# Autodesk Inventor assembly: s-assy-motor
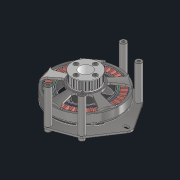
[picture p0: Inventor's stored thumbnail of the model, 180x180]
Saved by Autodesk Inventor 2021 (Build 250183000, 183)
## iProperties
Created: 2021-07-12
Part Number: s-assy-motor
Document SubType Name: Assembly
Designer: yuta0
Mass: 337.358 g
Surface Area: 828.401 cm^2
Volume: 95.8223 cm^3
Density: 3.52066 g/cm^3
Author: yuta0
## Documents named in this file (9)
- C:\Users\yuta0\Documents\GitHub\catchrobo_hardware\assy-robot\s-assy-motor.iam
- C:\Users\yuta0\Documents\GitHub\catchrobo_hardware\assy-robot\ex8108.iam
- C:\Users\yuta0\Documents\GitHub\catchrobo_hardware\assy-robot\CBSTNR3-12.ipt
- C:\Users\yuta0\Documents\GitHub\catchrobo_hardware\assy-robot\s-assy-unit-magnet.iam
- C:\Users\yuta0\Documents\GitHub\catchrobo_hardware\assy-robot\s-assy-unit-encoder.iam
- C:\Users\yuta0\Documents\GitHub\catchrobo_hardware\assy-robot\CB4-6.ipt
- C:\Users\yuta0\Documents\GitHub\catchrobo_hardware\assy-robot\base42.ipt
- C:\Users\yuta0\Documents\GitHub\catchrobo_hardware\assy-robot\ARF-445.ipt
- C:\Users\yuta0\Documents\GitHub\catchrobo_hardware\assy-robot\steel_plate7.ipt
## Components (21 placed, 8 different names)
1. s-assy-unit-magnet:1 [sub-assembly] — メイト:6, メイト:40, メイト:43
2. s-assy-unit-encoder:1 [sub-assembly] — メイト:43, メイト:46, メイト:65
3. ex8108:2 [sub-assembly] — メイト:12, メイト:33, メイト:36, メイト:42, メイト:63, メイト:64
4. base42:1 — メイト:33, メイト:36, メイト:37, メイト:38, メイト:39, メイト:63
5. CB4-6:1 — メイト:55, メイト:56
6. ARF-445:2 — メイト:47, メイト:48
7. steel_plate7:1 — メイト:40, メイト:42, メイト:45, メイト:46, メイト:47, メイト:48, メイト:49, メイト:50, メイト:51, メイト:52, メイト:53, メイト:54, メイト:55, メイト:56, メイト:57, メイト:58, メイト:59, メイト:60, メイト:61, メイト:62, メイト:64
8. ARF-445:1 — メイト:49, メイト:50
9. ARF-445:3 — メイト:51, メイト:52
10. ARF-445:4 — メイト:53, メイト:54
11. CB4-6:3 — メイト:57, メイト:58
12. CB4-6:4 — メイト:59, メイト:60
13. CB4-6:5 — メイト:61, メイト:62
14. CB4-6:2 — メイト:45
15. CBSTNR3-12:1 — メイト:37, メイト:38, メイト:39
16. CB4-6:6 — メイト:65
17. CBSTNR3-12:2
18. CB4-6:7
19. CBSTNR3-12:3
20. CB4-6:8
21. CBSTNR3-12:4
## Component patterns: (4 elements, first: CB4-6:2 + CBSTNR3-12:1)
## Relationships (31: Mate 31)
- メイト:6 [Mate]: s-assy-unit-magnet:1
- メイト:12 [Mate]: ex8108:2
- メイト:33 [Mate]: ex8108:2 ↔ base42:1
- メイト:36 [Mate]: ex8108:2 ↔ base42:1
- メイト:37 [Mate]: base42:1 ↔ CBSTNR3-12:1
- メイト:38 [Mate]: base42:1 ↔ CBSTNR3-12:1
- メイト:39 [Mate]: base42:1 ↔ CBSTNR3-12:1
- メイト:40 [Mate]: s-assy-unit-magnet:1 ↔ steel_plate7:1
- メイト:42 [Mate]: ex8108:2 ↔ steel_plate7:1
- メイト:43 [Mate]: s-assy-unit-magnet:1 ↔ s-assy-unit-encoder:1
- メイト:45 [Mate]: steel_plate7:1 ↔ CB4-6:2
- メイト:46 [Mate]: s-assy-unit-encoder:1 ↔ steel_plate7:1
- メイト:47 [Mate]: ARF-445:2 ↔ steel_plate7:1
- メイト:48 [Mate]: ARF-445:2 ↔ steel_plate7:1
- メイト:49 [Mate]: steel_plate7:1 ↔ ARF-445:1
- メイト:50 [Mate]: steel_plate7:1 ↔ ARF-445:1
- メイト:51 [Mate]: steel_plate7:1 ↔ ARF-445:3
- メイト:52 [Mate]: steel_plate7:1 ↔ ARF-445:3
- メイト:53 [Mate]: steel_plate7:1 ↔ ARF-445:4
- メイト:54 [Mate]: steel_plate7:1 ↔ ARF-445:4
- メイト:55 [Mate]: CB4-6:1 ↔ steel_plate7:1
- メイト:56 [Mate]: CB4-6:1 ↔ steel_plate7:1
- メイト:57 [Mate]: steel_plate7:1 ↔ CB4-6:3
- メイト:58 [Mate]: steel_plate7:1 ↔ CB4-6:3
- メイト:59 [Mate]: steel_plate7:1 ↔ CB4-6:4
- メイト:60 [Mate]: steel_plate7:1 ↔ CB4-6:4
- メイト:61 [Mate]: steel_plate7:1 ↔ CB4-6:5
- メイト:62 [Mate]: steel_plate7:1 ↔ CB4-6:5
- メイト:63 [Mate]: ex8108:2 ↔ base42:1
- メイト:64 [Mate]: ex8108:2 ↔ steel_plate7:1
- メイト:65 [Mate]: s-assy-unit-encoder:1 ↔ CB4-6:6
